# Autodesk Inventor assembly: obj6
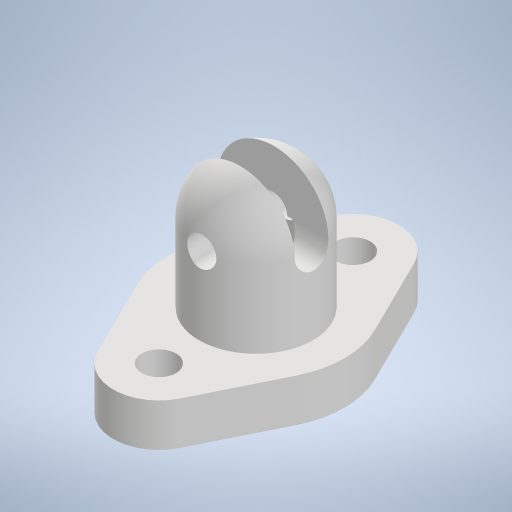
[picture p0: Inventor's stored thumbnail of the model, 512x512]
Saved by Autodesk Inventor 2023.2 (Build 272271030, 271C)
## iProperties
Created: 2023-02-25
Part Number: obj6
Document SubType Name: Assembly
Designer: Cris Pat
Author: Cris Pat
## Documents named in this file (3)
- C:\Users\Cris Pat\Desktop\U\Semestre 9\disenio e innovacion\CAD\obj6.iam
- C:\Users\Cris Pat\Desktop\U\Semestre 9\disenio e innovacion\CAD\cupula_obj5.ipt
- C:\Users\Cris Pat\Desktop\U\Semestre 9\disenio e innovacion\CAD\base_obj5.ipt
## Components (2 placed, 2 different names)
1. cupula_obj5:1 — Rigid:1
2. base_obj5:1 — Rigid:1
## Relationships (1: WeldJoint 1)
- Rigid:1 [WeldJoint]: cupula_obj5:1 ↔ base_obj5:1
